# Autodesk Inventor assembly: 3-6V DC Gearbox Electromotor
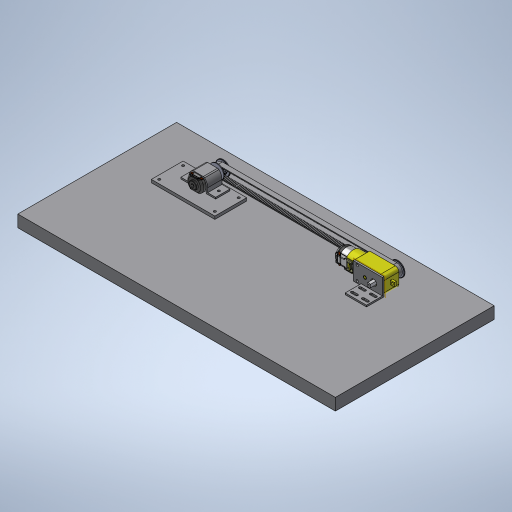
[picture p0: Inventor's stored thumbnail of the model, 512x512]
Saved by Autodesk Inventor 2023 (Build 270158000, 158)
## iProperties
Created: 2020-10-25
Part Number: 3-6V DC Gearbox Electromotor
Document SubType Name: Assembly
Designer: Niels
Author: Niels
## Documents named in this file (9)
- C:\Users\klebe\OneDrive\Área de Trabalho\esteira\motor\3-6V DC Gearbox Electromotor.iam
- C:\Users\klebe\OneDrive\Área de Trabalho\esteira\motor\DC 3-6V Gearbox Motor.ipt
- C:\Users\klebe\OneDrive\Área de Trabalho\esteira\motor\3V DC Electromotor.ipt
- C:\Users\klebe\OneDrive\Área de Trabalho\esteira\motor\Part3 - Gearbox.ipt
- C:\Users\klebe\OneDrive\Área de Trabalho\esteira\polia\Rolamento Gt20.ipt
- C:\Users\klebe\OneDrive\Área de Trabalho\esteira\esteira\esteira_correia.ipt
- C:\Users\klebe\OneDrive\Área de Trabalho\esteira\Base\base1.ipt
- C:\Users\klebe\OneDrive\Área de Trabalho\esteira\suporte\suporte_motor_amarelo.ipt
- C:\Users\klebe\OneDrive\Área de Trabalho\esteira\suporte\suporte_motor_1.ipt
## Components (10 placed, 8 different names)
1. DC 3-6V Gearbox Motor:1 — Insert:1, Mate:1, Flush:1, Rotational:1, Flush:4, Flush:7
2. 3V DC Electromotor:1 — Insert:1, Mate:1
3. Part3 - Gearbox:1 — Flush:2
4. Rolamento Gt20:2 — Rotational:1, Flush:3, Rotational:2
5. esteira_correia:1 — Flush:3, Rotational:2, Rotational:3
6. 3V DC Electromotor:2 — Rigid:1, Flush:9
7. Rolamento Gt20:3 — Rotational:3, Rigid:1
8. base1:1 — Flush:4, Flush:5, Flush:8
9. suporte_motor_amarelo:1 — Flush:5, Flush:7
10. suporte_motor_1:1 — Flush:8, Flush:9
## Relationships (14: Flush 8, RevoluteJoint 3, Insert 1, Mate 1, WeldJoint 1)
- Insert:1: DC 3-6V Gearbox Motor:1 ↔ 3V DC Electromotor:1
- Mate:1 (0.15 mm): DC 3-6V Gearbox Motor:1 ↔ 3V DC Electromotor:1
- Flush:1 (-3 mm): DC 3-6V Gearbox Motor:1
- Flush:2: Part3 - Gearbox:1
- Rotational:1 [RevoluteJoint] (2 mm): DC 3-6V Gearbox Motor:1 ↔ Rolamento Gt20:2
- Flush:3: Rolamento Gt20:2 ↔ esteira_correia:1
- Rotational:2 [RevoluteJoint] (1.25 mm): Rolamento Gt20:2 ↔ esteira_correia:1
- Rotational:3 [RevoluteJoint] (1.25 mm): esteira_correia:1 ↔ Rolamento Gt20:3
- Rigid:1 [WeldJoint] (1 mm): 3V DC Electromotor:2 ↔ Rolamento Gt20:3
- Flush:4: DC 3-6V Gearbox Motor:1 ↔ base1:1
- Flush:5: base1:1 ↔ suporte_motor_amarelo:1
- Flush:7: DC 3-6V Gearbox Motor:1 ↔ suporte_motor_amarelo:1
- Flush:8: base1:1 ↔ suporte_motor_1:1
- Flush:9: 3V DC Electromotor:2 ↔ suporte_motor_1:1
